# Autodesk Inventor assembly: 811001-X1 & 811000 & 810500_Robot Shield & Quickstart & Shield Standoff Kit ASSY
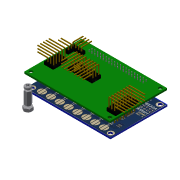
[picture p0: Inventor's stored thumbnail of the model, 180x180]
Saved by Autodesk Inventor 2015 (Build 190159000, 159)
## iProperties
Created: 2014-08-02
Part Number: 811001-X1 & 811000 & 810500_Robot Shield & Quickstart & Shield Standoff Kit ASSY
Document SubType Name: Assembly
Designer: david
Author: david
## Documents named in this file (6)
- C:\SharedDrive\Dropbox\FAST Robotics\Products\810001_FAST Robot Shield\CAD\810001_FAST Robot Shield\811001-X1 & 811000 & 810500_Robot Shield & Quickstart & Shield Standoff Kit ASSY.iam
- C:\SharedDrive\Dropbox\FAST Robotics\Products\810001_FAST Robot Shield\CAD\810001_FAST Robot Shield\810001-X1.iam
- C:\SharedDrive\Dropbox\FAST Robotics\Products\811000_Parallax Quickstart\CAD\811000_Parallax Quickstart\811000_Parallax Quickstart ASSY.iam
- C:\SharedDrive\Dropbox\FAST Robotics\Products\810500_Shield Standoff Kit - .4375in\CAD\Imported Components\500503\500503.ipt
- C:\SharedDrive\Dropbox\FAST Robotics\Products\810500_Shield Standoff Kit - .4375in\CAD\Imported Components\500504\500504.ipt
- C:\SharedDrive\Dropbox\FAST Robotics\Products\810500_Shield Standoff Kit - .4375in\CAD\Imported Components\525500\525500.ipt
## Components (5 placed, 5 different names)
1. 810001-X1:1 [sub-assembly] — Mate:2, Angle:1
2. 811000_Parallax Quickstart ASSY:1 [sub-assembly] — Mate:2, Angle:1
3. 500503:2 — Insert:5
4. 500504:2 — Insert:4
5. 525500:2 — Insert:4, Insert:5
## Relationships (4: Insert 2, Mate 1, Angle 1)
- Mate:2: 810001-X1:1 ↔ 811000_Parallax Quickstart ASSY:1
- Angle:1 (0 deg): 810001-X1:1 ↔ 811000_Parallax Quickstart ASSY:1
- Insert:4 (1.524 mm): 500504:2 ↔ 525500:2
- Insert:5 (1.524 mm): 500503:2 ↔ 525500:2
